# Autodesk Inventor assembly: front-left
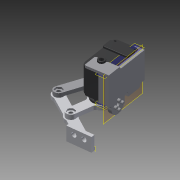
[picture p0: Inventor's stored thumbnail of the model, 180x180]
Saved by Autodesk Inventor 2014 (Build 180170000, 170)
## iProperties
Created: 2015-05-23
Part Number: front-left
Document SubType Name: Assembly
Designer: Hideyuki Takei
Author: Hideyuki Takei
## Documents named in this file (7)
- C:\Users\hide\Desktop\soth-bonsai\cad\front-left.iam
- C:\Users\hide\Desktop\soth-bonsai\cad\RS304md-simple.ipt
- C:\Users\hide\Desktop\soth-bonsai\cad\RS304MD-ServoHorn.ipt
- C:\Users\hide\Desktop\soth-bonsai\cad\leg_MIR.ipt
- C:\Users\hide\Desktop\soth-bonsai\cad\servo-holder_MIR.ipt
- C:\Users\hide\Desktop\soth-bonsai\cad\link-long.ipt
- C:\Users\hide\Desktop\soth-bonsai\cad\link-short.ipt
## Components (6 placed, 6 different names)
1. RS304md-simple:1 — メイト:4, メイト:5, メイト:6, メイト:7, メイト:8, メイト:12
2. RS304MD-ServoHorn:1 — メイト:4, メイト:5, メイト:9
3. leg_MIR:1 — メイト:13, メイト:14, メイト:15, メイト:16
4. servo-holder_MIR:1 — メイト:6, メイト:7, メイト:8, メイト:10, メイト:11
5. link-long:1 — メイト:10, メイト:11, メイト:14, メイト:15
6. link-short:1 — メイト:9, メイト:12, メイト:13, メイト:16
## Relationships (13: Mate 13)
- メイト:4 [Mate]: RS304md-simple:1 ↔ RS304MD-ServoHorn:1
- メイト:5 [Mate]: RS304md-simple:1 ↔ RS304MD-ServoHorn:1
- メイト:6 [Mate]: RS304md-simple:1 ↔ servo-holder_MIR:1
- メイト:7 [Mate]: RS304md-simple:1 ↔ servo-holder_MIR:1
- メイト:8 [Mate]: RS304md-simple:1 ↔ servo-holder_MIR:1
- メイト:9 [Mate]: RS304MD-ServoHorn:1 ↔ link-short:1
- メイト:10 [Mate]: servo-holder_MIR:1 ↔ link-long:1
- メイト:11 [Mate]: servo-holder_MIR:1 ↔ link-long:1
- メイト:12 [Mate]: RS304md-simple:1 ↔ link-short:1
- メイト:13 [Mate]: leg_MIR:1 ↔ link-short:1
- メイト:14 [Mate]: leg_MIR:1 ↔ link-long:1
- メイト:15 [Mate]: leg_MIR:1 ↔ link-long:1
- メイト:16 [Mate]: leg_MIR:1 ↔ link-short:1
